# Autodesk Inventor assembly: MecanumWheelFullForVexmotor
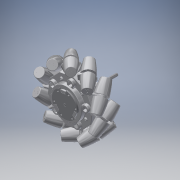
[picture p0: Inventor's stored thumbnail of the model, 180x180]
Saved by Autodesk Inventor 2017 (Build 210142000, 142)
## iProperties
Created: 2017-12-02
Part Number: MecanumWheelFullForVexmotor
Document SubType Name: Assembly
Designer: User
Author: User
## Documents named in this file (6)
- C:\Robotics\CAD\2017-18_CAD\Prototypes\MecanumWheelFullForVexmotor.iam
- C:\Robotics\CAD\COTSParts\Vex\6inchMecanumRight217-2586-STEP\6inchMecanumRight217-2586.20121203.ipt
- C:\Robotics\CAD\COTSParts\Vex\VersaHub.5inchBore217-4009-STEP-20140807\VersaHub.5inchBore217-4009-STEP-20140807.ipt
- C:\Robotics\CAD\COTSParts\Rev\REV-41-1147HexHub.ipt
- C:\Robotics\CAD\COTSParts\Rev\REV-41-1349.ipt
- C:\Robotics\CAD\2017-18_CAD\Prototypes\NewMechanumWheelHub.ipt
## Components (6 placed, 5 different names)
1. 6inchMecanumRight217-2586.20121203:1 — Mate:1, Mate:2, Mate:3, Mate:4, Mate:5, Mate:6, Mate:10, Mate:18, Mate:19
2. VersaHub.5inchBore217-4009-STEP-20140807:1 — Mate:1, Mate:2, Mate:3, Mate:9, Mate:14
3. VersaHub.5inchBore217-4009-STEP-20140807:2 — Mate:4, Mate:5, Mate:6, Flush:2
4. REV-41-1147HexHub:2 — Mate:9, Mate:10, Mate:12, Mate:13, Mate:14
5. REV-41-1349:1 — Flush:2, Mate:12, Mate:13, Mate:17
6. NewMechanumWheelHub:1 — Mate:17, Mate:18, Mate:19
## Relationships (15: Mate 14, Flush 1)
- Mate:1: 6inchMecanumRight217-2586.20121203:1 ↔ VersaHub.5inchBore217-4009-STEP-20140807:1
- Mate:2: 6inchMecanumRight217-2586.20121203:1 ↔ VersaHub.5inchBore217-4009-STEP-20140807:1
- Mate:3: 6inchMecanumRight217-2586.20121203:1 ↔ VersaHub.5inchBore217-4009-STEP-20140807:1
- Mate:4: 6inchMecanumRight217-2586.20121203:1 ↔ VersaHub.5inchBore217-4009-STEP-20140807:2
- Mate:5: 6inchMecanumRight217-2586.20121203:1 ↔ VersaHub.5inchBore217-4009-STEP-20140807:2
- Mate:6: 6inchMecanumRight217-2586.20121203:1 ↔ VersaHub.5inchBore217-4009-STEP-20140807:2
- Flush:2: VersaHub.5inchBore217-4009-STEP-20140807:2 ↔ REV-41-1349:1
- Mate:9: VersaHub.5inchBore217-4009-STEP-20140807:1 ↔ REV-41-1147HexHub:2
- Mate:10: 6inchMecanumRight217-2586.20121203:1 ↔ REV-41-1147HexHub:2
- Mate:12: REV-41-1147HexHub:2 ↔ REV-41-1349:1
- Mate:13: REV-41-1147HexHub:2 ↔ REV-41-1349:1
- Mate:14: VersaHub.5inchBore217-4009-STEP-20140807:1 ↔ REV-41-1147HexHub:2
- Mate:17: REV-41-1349:1 ↔ NewMechanumWheelHub:1
- Mate:18: 6inchMecanumRight217-2586.20121203:1 ↔ NewMechanumWheelHub:1
- Mate:19: 6inchMecanumRight217-2586.20121203:1 ↔ NewMechanumWheelHub:1
